# Autodesk Inventor assembly: 2220_Main Copper Box_V1
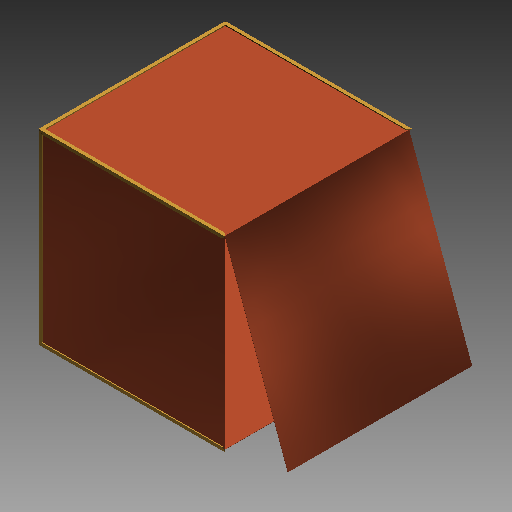
[picture p0: Inventor's stored thumbnail of the model, 512x512]
Saved by Autodesk Inventor 2020 (Build 240168000, 168)
## iProperties
Created: 2017-08-01
Part Number: 2220_Main Copper Box_V1
Document SubType Name: Assembly
Designer: MPI
Author: MPI
## Documents named in this file (6)
- C:\Users\RFLab\Dropbox\MPI Group Folder\fMPI (Rodent)\Small Bore Imager_Open Source Files\Inventor Files\2xxx_Stationary Structure\22xx_Electrical Shielding\2220_Main Copper Box_V1.iam
- C:\Users\RFLab\Dropbox\MPI Group Folder\fMPI (Rodent)\Small Bore Imager_Open Source Files\Inventor Files\2xxx_Stationary Structure\22xx_Electrical Shielding\222x_Main Copper Box\2221_Copper Box Side_V1.ipt
- C:\Users\RFLab\Dropbox\MPI Group Folder\fMPI (Rodent)\Small Bore Imager_Open Source Files\Inventor Files\2xxx_Stationary Structure\22xx_Electrical Shielding\222x_Main Copper Box\2221A_Copper Box Side_Hole_V1.ipt
- C:\Users\RFLab\Dropbox\MPI Group Folder\fMPI (Rodent)\Small Bore Imager_Open Source Files\Inventor Files\2xxx_Stationary Structure\22xx_Electrical Shielding\222x_Main Copper Box\2221B_Copper Box Side_Feedthrough_V1.ipt
- C:\Users\RFLab\Dropbox\MPI Group Folder\fMPI (Rodent)\Small Bore Imager_Open Source Files\Inventor Files\2xxx_Stationary Structure\22xx_Electrical Shielding\222x_Main Copper Box\2221C_BNC Feedthrough_V1.ipt
- C:\Users\RFLab\Dropbox\MPI Group Folder\fMPI (Rodent)\Small Bore Imager_Open Source Files\Inventor Files\2xxx_Stationary Structure\22xx_Electrical Shielding\222x_Main Copper Box\2222_Brass Angle Bracket_V1.ipt
## Components (19 placed, 5 different names)
1. 2221_Copper Box Side_V1:7 — Mate:2, Mate:3, Angle:2, Mate:56, Mate:60, Mate:66
2. 2221A_Copper Box Side_Hole_V1:2 — Flush:7, Flush:8, Mate:49, Mate:52, Mate:59, Mate:62
3. 2221_Copper Box Side_V1:3 — Mate:2, Mate:3, Mate:47, Mate:48, Flush:17, Mate:63, Mate:65, Mate:68, Symmetry:1
4. 2221B_Copper Box Side_Feedthrough_V1:1 — Flush:7, Mate:34, Mate:41, Mate:42, Mate:43, Mate:44, Mate:45, Mate:46, Mate:50, Mate:57, Symmetry:1
5. 2222_Brass Angle Bracket_V1:1 — Mate:52, Mate:53, Mate:54, Mate:55, Mate:70
6. 2221_Copper Box Side_V1:6 — Flush:8, Mate:53, Mate:69
7. 2221_Copper Box Side_V1:5 — Mate:47, Angle:2, Mate:48, Flush:17
8. 2222_Brass Angle Bracket_V1:2 — Mate:34, Mate:51, Mate:55
9. 2221C_BNC Feedthrough_V1:1 — Flush:12, Flush:13, Mate:41, Mate:42
10. 2221C_BNC Feedthrough_V1:2 — Flush:11, Flush:12, Flush:13, Flush:14, Mate:46
11. 2221C_BNC Feedthrough_V1:3 — Flush:9, Flush:10, Flush:11, Flush:14, Flush:15, Mate:45
12. 2221C_BNC Feedthrough_V1:4 — Flush:9, Flush:15, Flush:16, Mate:43
13. 2221C_BNC Feedthrough_V1:5 — Flush:10, Flush:16, Mate:44
14. 2222_Brass Angle Bracket_V1:3 — Mate:49, Mate:50, Mate:51, Mate:54, Mate:58
15. 2222_Brass Angle Bracket_V1:4 — Mate:56, Mate:57, Mate:58, Mate:61
16. 2222_Brass Angle Bracket_V1:5 — Mate:59, Mate:60, Mate:61, Mate:64, Mate:67
17. 2222_Brass Angle Bracket_V1:6 — Mate:62, Mate:63, Mate:64
18. 2222_Brass Angle Bracket_V1:7 — Mate:65, Mate:66, Mate:67
19. 2222_Brass Angle Bracket_V1:8 — Mate:68, Mate:69, Mate:70
## Relationships (54: Mate 39, Flush 12, Angle 2, Symmetry 1)
- [Mate]: 2221_Copper Box Side_V1:7 ↔ 2221A_Copper Box Side_Hole_V1:2
- [Angle] (270 deg): 2221_Copper Box Side_V1:7 ↔ 2221A_Copper Box Side_Hole_V1:2
- [Flush]: 2221_Copper Box Side_V1:7 ↔ 2221A_Copper Box Side_Hole_V1:2
- Mate:2: 2221_Copper Box Side_V1:7 ↔ 2221_Copper Box Side_V1:3
- Mate:3: 2221_Copper Box Side_V1:7 ↔ 2221_Copper Box Side_V1:3
- [Mate]: 2221A_Copper Box Side_Hole_V1:2 ↔ 2221_Copper Box Side_V1:3
- [Mate]: 2221A_Copper Box Side_Hole_V1:2 ↔ 2221B_Copper Box Side_Feedthrough_V1:1
- Flush:7: 2221A_Copper Box Side_Hole_V1:2 ↔ 2221B_Copper Box Side_Feedthrough_V1:1
- [Mate]: 2221_Copper Box Side_V1:3 ↔ 2221_Copper Box Side_V1:6
- [Mate]: 2221_Copper Box Side_V1:3 ↔ 2221_Copper Box Side_V1:6
- [Mate]: 2221_Copper Box Side_V1:6 ↔ 2222_Brass Angle Bracket_V1:2
- Mate:34: 2221B_Copper Box Side_Feedthrough_V1:1 ↔ 2222_Brass Angle Bracket_V1:2
- Flush:8: 2221A_Copper Box Side_Hole_V1:2 ↔ 2221_Copper Box Side_V1:6
- Flush:9: 2221C_BNC Feedthrough_V1:3 ↔ 2221C_BNC Feedthrough_V1:4
- Flush:10: 2221C_BNC Feedthrough_V1:3 ↔ 2221C_BNC Feedthrough_V1:5
- Flush:11: 2221C_BNC Feedthrough_V1:2 ↔ 2221C_BNC Feedthrough_V1:3
- Flush:12: 2221C_BNC Feedthrough_V1:1 ↔ 2221C_BNC Feedthrough_V1:2
- Flush:13: 2221C_BNC Feedthrough_V1:1 ↔ 2221C_BNC Feedthrough_V1:2
- Flush:14: 2221C_BNC Feedthrough_V1:2 ↔ 2221C_BNC Feedthrough_V1:3
- Flush:15: 2221C_BNC Feedthrough_V1:3 ↔ 2221C_BNC Feedthrough_V1:4
- Flush:16: 2221C_BNC Feedthrough_V1:4 ↔ 2221C_BNC Feedthrough_V1:5
- Mate:41: 2221B_Copper Box Side_Feedthrough_V1:1 ↔ 2221C_BNC Feedthrough_V1:1
- Mate:42: 2221B_Copper Box Side_Feedthrough_V1:1 ↔ 2221C_BNC Feedthrough_V1:1
- Mate:43: 2221B_Copper Box Side_Feedthrough_V1:1 ↔ 2221C_BNC Feedthrough_V1:4
- Mate:44: 2221B_Copper Box Side_Feedthrough_V1:1 ↔ 2221C_BNC Feedthrough_V1:5
- Mate:45: 2221B_Copper Box Side_Feedthrough_V1:1 ↔ 2221C_BNC Feedthrough_V1:3
- Mate:46: 2221B_Copper Box Side_Feedthrough_V1:1 ↔ 2221C_BNC Feedthrough_V1:2
- Mate:47: 2221_Copper Box Side_V1:3 ↔ 2221_Copper Box Side_V1:5
- Angle:2 (200 deg): 2221_Copper Box Side_V1:7 ↔ 2221_Copper Box Side_V1:5
- Mate:48: 2221_Copper Box Side_V1:3 ↔ 2221_Copper Box Side_V1:5
- Flush:17: 2221_Copper Box Side_V1:3 ↔ 2221_Copper Box Side_V1:5
- Mate:49: 2221A_Copper Box Side_Hole_V1:2 ↔ 2222_Brass Angle Bracket_V1:3
- Mate:50: 2221B_Copper Box Side_Feedthrough_V1:1 ↔ 2222_Brass Angle Bracket_V1:3
- Mate:51: 2222_Brass Angle Bracket_V1:2 ↔ 2222_Brass Angle Bracket_V1:3
- Mate:52: 2221A_Copper Box Side_Hole_V1:2 ↔ 2222_Brass Angle Bracket_V1:1
- Mate:53: 2222_Brass Angle Bracket_V1:1 ↔ 2221_Copper Box Side_V1:6
- Mate:54: 2222_Brass Angle Bracket_V1:1 ↔ 2222_Brass Angle Bracket_V1:3
- Mate:55: 2222_Brass Angle Bracket_V1:1 ↔ 2222_Brass Angle Bracket_V1:2
- Mate:56: 2221_Copper Box Side_V1:7 ↔ 2222_Brass Angle Bracket_V1:4
- Mate:57: 2221B_Copper Box Side_Feedthrough_V1:1 ↔ 2222_Brass Angle Bracket_V1:4
- Mate:58: 2222_Brass Angle Bracket_V1:3 ↔ 2222_Brass Angle Bracket_V1:4
- Mate:59: 2221A_Copper Box Side_Hole_V1:2 ↔ 2222_Brass Angle Bracket_V1:5
- Mate:60: 2221_Copper Box Side_V1:7 ↔ 2222_Brass Angle Bracket_V1:5
- Mate:61: 2222_Brass Angle Bracket_V1:4 ↔ 2222_Brass Angle Bracket_V1:5
- Mate:62: 2221A_Copper Box Side_Hole_V1:2 ↔ 2222_Brass Angle Bracket_V1:6
- Mate:63: 2221_Copper Box Side_V1:3 ↔ 2222_Brass Angle Bracket_V1:6
- Mate:64: 2222_Brass Angle Bracket_V1:5 ↔ 2222_Brass Angle Bracket_V1:6
- Mate:65: 2221_Copper Box Side_V1:3 ↔ 2222_Brass Angle Bracket_V1:7
- Mate:66: 2221_Copper Box Side_V1:7 ↔ 2222_Brass Angle Bracket_V1:7
- Mate:67: 2222_Brass Angle Bracket_V1:5 ↔ 2222_Brass Angle Bracket_V1:7
- Mate:68: 2221_Copper Box Side_V1:3 ↔ 2222_Brass Angle Bracket_V1:8
- Mate:69: 2221_Copper Box Side_V1:6 ↔ 2222_Brass Angle Bracket_V1:8
- Mate:70: 2222_Brass Angle Bracket_V1:1 ↔ 2222_Brass Angle Bracket_V1:8
- Symmetry:1: 2221_Copper Box Side_V1:3 ↔ 2221B_Copper Box Side_Feedthrough_V1:1
